# Autodesk Inventor assembly: trigger_mechanism
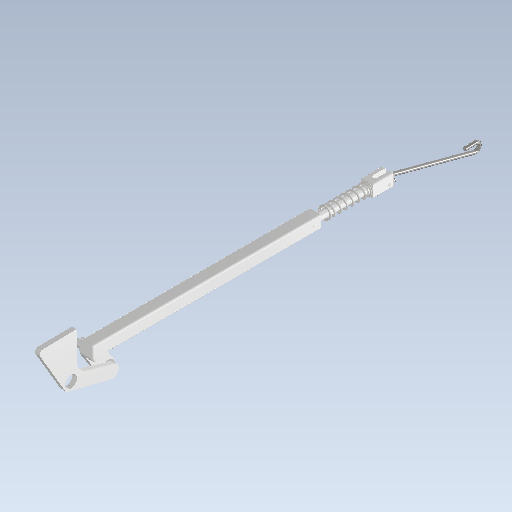
[picture p0: Inventor's stored thumbnail of the model, 512x512]
Saved by Autodesk Inventor 2021 (Build 250183000, 183)
## iProperties
Created: 2023-08-11
Part Number: trigger_mechanism
Document SubType Name: Weldment
Designer: Sergio
Weld Material: Welded Aluminum-6061
Author: Sergio
## Documents named in this file (7)
- D:\Sergio\OneDrive - Escuela Superior Politécnica del Litoral\Documentos\12vo Semestre (último)\Diseño Mecatrónico\Proyecto\Diseño Mecánico\solucion GANADORA\trigger_mechanism\Mecanismo de Gatillo.iam
- D:\Sergio\OneDrive - Escuela Superior Politécnica del Litoral\Documentos\12vo Semestre (último)\Diseño Mecatrónico\Proyecto\Diseño Mecánico\solucion GANADORA\trigger_mechanism\Gatillo.ipt
- D:\Sergio\OneDrive - Escuela Superior Politécnica del Litoral\Documentos\12vo Semestre (último)\Diseño Mecatrónico\Proyecto\Diseño Mecánico\solucion GANADORA\trigger_mechanism\Eslabón 3.ipt
- D:\Sergio\OneDrive - Escuela Superior Politécnica del Litoral\Documentos\12vo Semestre (último)\Diseño Mecatrónico\Proyecto\Diseño Mecánico\solucion GANADORA\trigger_mechanism\link\Eslabón conector.iam
- D:\Sergio\OneDrive - Escuela Superior Politécnica del Litoral\Documentos\12vo Semestre (último)\Diseño Mecatrónico\Proyecto\Diseño Mecánico\solucion GANADORA\trigger_mechanism\Pasador de eslabón.ipt
- D:\Sergio\OneDrive - Escuela Superior Politécnica del Litoral\Documentos\12vo Semestre (último)\Diseño Mecatrónico\Proyecto\Diseño Mecánico\solucion GANADORA\trigger_mechanism\Varilla Gancho.ipt
- D:\Sergio\OneDrive - Escuela Superior Politécnica del Litoral\Documentos\12vo Semestre (último)\Diseño Mecatrónico\Proyecto\Diseño Mecánico\solucion GANADORA\parameters.xlsx
## Components (5 placed, 5 different names)
1. Gatillo:1 — Tangente:2, Coincidencia:1
2. Eslabón 3:1 — Tangente:2, Coincidencia:1, Coincidencia:2, Coincidencia:3
3. Eslabón conector:1 [sub-assembly] — Coincidencia:2, Coincidencia:3, Nivelación:5, Coincidencia:4, Coincidencia:5
4. Pasador de eslabón:1 — Coincidencia:4, Coincidencia:5, Tangente:3, Coincidencia:6
5. Varilla Gancho:1 — Tangente:3, Coincidencia:6
## Relationships (9: Mate 6, Tangent 2, Flush 1)
- Tangente:2: Gatillo:1 ↔ Eslabón 3:1
- Coincidencia:1 [Mate]: Gatillo:1 ↔ Eslabón 3:1
- Coincidencia:2 [Mate]: Eslabón 3:1 ↔ Eslabón conector:1
- Coincidencia:3 [Mate]: Eslabón 3:1 ↔ Eslabón conector:1
- Nivelación:5 [Flush]: Eslabón conector:1
- Coincidencia:4 [Mate]: Eslabón conector:1 ↔ Pasador de eslabón:1
- Coincidencia:5 [Mate]: Eslabón conector:1 ↔ Pasador de eslabón:1
- Tangente:3: Pasador de eslabón:1 ↔ Varilla Gancho:1
- Coincidencia:6 [Mate]: Pasador de eslabón:1 ↔ Varilla Gancho:1
## Named parameters: thikness = 2 mm, offset = 1 mm, r1 = 5.55 mm, r2o = 59.75 mm, delta_y = 6 mm, r4 = 60 mm, wire_d = 1 mm, vueltas = 4, width_ang_spring = 5 mm, spring_int_diam = 8.5 mm, spring_ext_diam = 10.5 mm, r3 = 8.25 mm, r3R = 4.75 mm, r3T = 6.74537 mm, alpha = 54.847297 deg, alpha2 = 270 deg, theta3 = 305.152703 deg, delta_theta_3 = 45 deg, joint_width = 12 mm, joint_radius = 7.75 mm, shaft_width = 15 mm, shaft_joint_diameter = 7.75 mm, separation_space = 0.5 mm, height_finger = 42 mm, width_finger = 20 mm, cell_screw_head_diameter = 4 mm, cell_screw_diameter = 2 mm, cell_space = 2 mm, cell_width = 6 mm, cell_theta_position = 60 deg, cell_thikness = 1 mm, cell_lenght = 37 mm, cell_z_space = 5 mm, secure_distance = 250 mm, hand_lenght = 110 mm, hand_space = 30 mm, wire_D = 2.3 mm, width_link = 8 mm, Dt = 1.05949 mm, Djoint_shaft = 2.3 mm, shaft_x = 1.45 mm, shaft_y = 6.45 mm, lenght_body_link = 186.05 mm, lenght_bar_support = 201.65 mm, trigger_offset = 2 mm, m2_theta2o = 107 deg, m2_r2 = 28 mm, e = 9 mm, So = 17 mm, m2_theta3o = -30 deg, m2_r3 = 19.75 mm, m2_delta_theta1 = 15 deg, m2_theta3f = -60 deg, trigger_thumb_lenght = 6 mm, width_r12 = 8 mm, width_r3 = 10 mm, m2_r1 = 25.2 mm, m2_r1_down_width = 20 mm, r3_thikness = 3.5 mm, t_thikness = 3 mm, t_thikness2 = 10 mm, tg_lenght = 30 mm, tg_width = 4 mm, pivot_screw_d = 4 mm, pivot_diameter = 7 mm, sj_diam_shaft = 6 mm, sj_groove = 2 mm, sj_groove_deep = 7 mm, sj_head_D = 7 mm, sj_head_d = 4.7464 mm, sj_head_height = 5 mm, theta3_recogido = 305.152703 deg, gj_d = 4 mm, gj_out_section = 6 mm, sf_head_height = 3 mm, screw_lenght = 12 mm, screwJ_top_D = 13 mm, sf_head_width = 4.5 mm, sf_head_grip_width = 2 mm, sf_thikness = 5 mm, sf_lenght = 9.5 mm, sf_head_angle = 45 deg, sf_base = 3 mm, screw_Dhead = 8 mm, gj_D = 6 mm, screwJ_base_D = 9 mm, screw_d = 4 mm, sf_head_offset = 0.25 mm, spring_lenght = 28 mm, spring_int_d = 6 mm, wire_spring_d = 1 mm, sfbox_theta1 = 60 deg, agarradera_theta = 60 deg, sfbox_theta2 = 45 deg, agarradera_position = 82.13077 mm, agarradera_width = 4 mm, thikness_box = 1.5 mm, box_slim_slider_lenght = 116 mm, flex_separation_theta = 60 deg, box_in_height = 35 mm, sf_flex_separation = 38.66667 mm, fat_width_slider = 2 mm, box_in_width = 72 mm, offset_base_box = 40 mm, int_width_slider = 2 mm, box_fat_slider_lenght = 67 mm, sfbox_width = 1.5 mm, box_base_width = 30 mm, box_separation = 10 mm, sfbox_tip_width = 2.5 mm, slim_width_slider = 1.5 mm, box_base_lenght = 120 mm, ext_width_slider = 3.5 mm, box_in_deep = 77 mm
